# Autodesk Inventor assembly: 68. Первичный вал
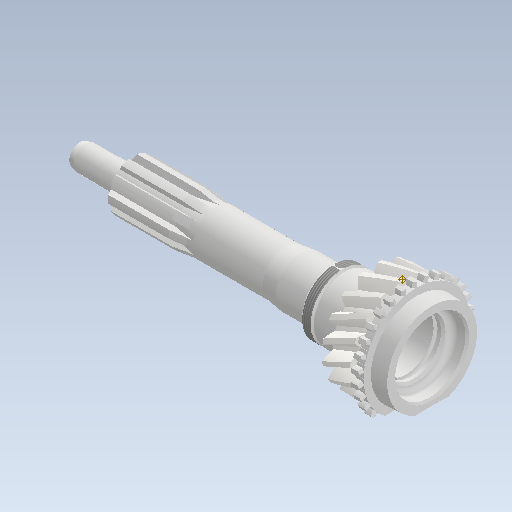
[picture p0: Inventor's stored thumbnail of the model, 512x512]
Saved by Autodesk Inventor 2021 (Build 250183000, 183)
## iProperties
Created: 2021-03-22
Part Number: 68. Первичный вал
Document SubType Name: Assembly
Designer: Данил
Author: Данил
## Documents named in this file (3)
- C:\Users\Данил\Desktop\Коробка передач\Детали\68. Первичный вал.iam
- C:\Users\Данил\Desktop\Коробка передач\Детали\68. Первичный вал.ipt
- C:\Users\Данил\Desktop\Коробка передач\Детали\68. Первичный вал\Мастер проектирования\Цилиндрическое зубчатое зацепление1.iam
## Components (2 placed, 2 different names)
1. 68. Первичный вал:1 — Совмещение:2, Совмещение:5, Совмещение:6, Совмещение:7
2. Цилиндрическое зубчатое зацепление:1 [sub-assembly] — Совмещение:2, Совмещение:3, Совмещение:5, Совмещение:7
## Relationships (5: Mate 5)
- Совмещение:2 [Mate]: 68. Первичный вал:1 ↔ Цилиндрическое зубчатое зацепление:1
- Совмещение:3 [Mate]: Цилиндрическое зубчатое зацепление:1
- Совмещение:5 [Mate]: 68. Первичный вал:1 ↔ Цилиндрическое зубчатое зацепление:1
- Совмещение:6 [Mate]: 68. Первичный вал:1
- Совмещение:7 [Mate]: 68. Первичный вал:1 ↔ Цилиндрическое зубчатое зацепление:1
